# Autodesk Inventor assembly: Wetterstation
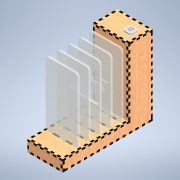
[picture p0: Inventor's stored thumbnail of the model, 180x180]
Saved by Autodesk Inventor 2021 (Build 250183000, 183)
## iProperties
Created: 2021-03-07
Part Number: Wetterstation
Document SubType Name: Assembly
Designer: Tilman
Author: Tilman
## Documents named in this file (16)
- C:\Users\Tilman\Desktop\UNI\Soft-Skills\Inventor\Wetterstation.iam
- C:\Users\Tilman\Desktop\UNI\Soft-Skills\Inventor\plate_top_middle.ipt
- C:\Users\Tilman\Desktop\UNI\Soft-Skills\Inventor\plate_front_small.ipt
- C:\Users\Tilman\Desktop\UNI\Soft-Skills\Inventor\plate_front_big.ipt
- C:\Users\Tilman\Desktop\UNI\Soft-Skills\Inventor\plate_top_small.ipt
- C:\Users\Tilman\Desktop\UNI\Soft-Skills\Inventor\plate_bottom.ipt
- C:\Users\Tilman\Desktop\UNI\Soft-Skills\Inventor\plate_back.ipt
- C:\Users\Tilman\Desktop\UNI\Soft-Skills\Inventor\plate_side.ipt
- C:\Users\Tilman\Desktop\UNI\Soft-Skills\Inventor\pane_cloud.ipt
- C:\Users\Tilman\Desktop\UNI\Soft-Skills\Inventor\plane_sun.ipt
- C:\Users\Tilman\Desktop\UNI\Soft-Skills\Inventor\plane_rain.ipt
- C:\Users\Tilman\Desktop\UNI\Soft-Skills\Inventor\pane.ipt
- C:\Users\Tilman\Desktop\UNI\Soft-Skills\Inventor\led_stand.ipt
- C:\Users\Tilman\Desktop\UNI\Soft-Skills\Inventor\pane_matt.ipt
- C:\Users\Tilman\Desktop\UNI\Soft-Skills\Inventor\ESP_stand.ipt
- C:\Users\Tilman\Desktop\UNI\Soft-Skills\Inventor\pane_stabilisor.ipt
## Components (16 placed, 15 different names)
1. plate_top_middle:1 — Starr:1, Starr:2, Starr:9, Starr:10, Starr:11, Starr:12, Starr:13
2. plate_front_small:1 — Starr:1, Starr:4, Starr:14
3. plate_front_big:1 — Starr:2, Starr:3
4. plate_top_small:1 — Starr:3, Passend:1
5. plate_bottom:1 — Starr:4, Starr:6, Starr:15, Passend:3, Passend:4
6. plate_back:1 — Starr:15
7. plate_side:1 — Starr:14, Passend:2
8. plate_side:2 — Starr:6
9. pane_cloud:1 — Starr:10
10. plane_sun:1 — Starr:11
11. plane_rain:1 — Starr:9
12. pane:1 — Starr:12, Passend:5, Passend:6
13. led_stand:1 — Passend:1
14. pane_matt:1 — Starr:13
15. ESP_stand:1 — Passend:2, Passend:3
16. pane_stabilisor:1 — Passend:4, Passend:5, Passend:6
## Relationships (18: WeldJoint 12, Mate 6)
- Starr:1 [WeldJoint]: plate_top_middle:1 ↔ plate_front_small:1
- Starr:2 [WeldJoint]: plate_top_middle:1 ↔ plate_front_big:1
- Starr:3 [WeldJoint]: plate_front_big:1 ↔ plate_top_small:1
- Starr:4 [WeldJoint]: plate_front_small:1 ↔ plate_bottom:1
- Starr:6 [WeldJoint]: plate_bottom:1 ↔ plate_side:2
- Starr:9 [WeldJoint]: plate_top_middle:1 ↔ plane_rain:1
- Starr:10 [WeldJoint]: plate_top_middle:1 ↔ pane_cloud:1
- Starr:11 [WeldJoint]: plate_top_middle:1 ↔ plane_sun:1
- Starr:12 [WeldJoint]: plate_top_middle:1 ↔ pane:1
- Passend:1 [Mate]: plate_top_small:1 ↔ led_stand:1
- Starr:13 [WeldJoint]: plate_top_middle:1 ↔ pane_matt:1
- Starr:14 [WeldJoint]: plate_front_small:1 ↔ plate_side:1
- Starr:15 [WeldJoint]: plate_bottom:1 ↔ plate_back:1
- Passend:2 [Mate]: plate_side:1 ↔ ESP_stand:1
- Passend:3 [Mate]: plate_bottom:1 ↔ ESP_stand:1
- Passend:4 [Mate]: plate_bottom:1 ↔ pane_stabilisor:1
- Passend:5 [Mate]: pane:1 ↔ pane_stabilisor:1
- Passend:6 [Mate]: pane:1 ↔ pane_stabilisor:1
